# Autodesk Inventor assembly: schunk_with_gripper_fingers
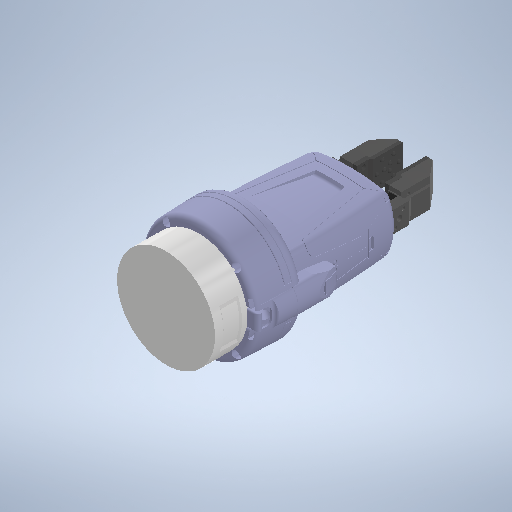
[picture p0: Inventor's stored thumbnail of the model, 512x512]
Saved by Autodesk Inventor 2025 (Build 290162010, 162A)
## iProperties
Created: 2024-08-06
Part Number: schunk_with_gripper_fingers
Document SubType Name: Assembly
Designer: caubeeluck
Author: caubeeluck
## Documents named in this file (21)
- D:\Projects\Archived\Misc\github\autoclean\AutoClean\cad_files\gripper\final_models\gripper_assembly_open\schunk_with_gripper_fingers.iam
- D:\Projects\Archived\Misc\github\autoclean\AutoClean\cad_files\gripper\final_models\gripper_assembly_open\schunk_with_gripper_fingers1.ipt
- D:\Projects\Archived\Misc\github\autoclean\AutoClean\cad_files\gripper\final_models\gripper_assembly_open\schunk_with_gripper_fingers2.ipt
- D:\Projects\Archived\Misc\github\autoclean\AutoClean\cad_files\gripper\final_models\gripper_assembly_open\schunk_with_gripper_fingers3.ipt
- D:\Projects\Archived\Misc\github\autoclean\AutoClean\cad_files\gripper\final_models\gripper_assembly_open\schunk_with_gripper_fingers4.ipt
- D:\Projects\Archived\Misc\github\autoclean\AutoClean\cad_files\gripper\final_models\gripper_assembly_open\schunk_with_gripper_fingers6.ipt
- D:\Projects\Archived\Misc\github\autoclean\AutoClean\cad_files\gripper\final_models\gripper_assembly_open\schunk_with_gripper_fingers7.ipt
- D:\Projects\Archived\Misc\github\autoclean\AutoClean\cad_files\gripper\final_models\gripper_assembly_open\schunk_with_gripper_fingers8.ipt
- D:\Projects\Archived\Misc\github\autoclean\AutoClean\cad_files\gripper\final_models\gripper_assembly_open\schunk_with_gripper_fingers9.ipt
- D:\Projects\Archived\Misc\github\autoclean\AutoClean\cad_files\gripper\final_models\gripper_assembly_open\schunk_with_gripper_fingers10.ipt
- D:\Projects\Archived\Misc\github\autoclean\AutoClean\cad_files\gripper\final_models\gripper_assembly_open\schunk_with_gripper_fingers11.ipt
- D:\Projects\Archived\Misc\github\autoclean\AutoClean\cad_files\gripper\final_models\gripper_assembly_open\schunk_with_gripper_fingers12.ipt
- D:\Projects\Archived\Misc\github\autoclean\AutoClean\cad_files\gripper\final_models\gripper_assembly_open\schunk_with_gripper_fingers13.ipt
- D:\Projects\Archived\Misc\github\autoclean\AutoClean\cad_files\gripper\final_models\gripper_assembly_open\schunk_with_gripper_fingers14.ipt
- D:\Projects\Archived\Misc\github\autoclean\AutoClean\cad_files\gripper\final_models\gripper_assembly_open\schunk_with_gripper_fingers15.ipt
- D:\Projects\Archived\Misc\github\autoclean\AutoClean\cad_files\gripper\final_models\gripper_assembly_open\schunk_with_gripper_fingers16.ipt
- D:\Projects\Archived\Misc\github\autoclean\AutoClean\cad_files\gripper\final_models\gripper_assembly_open\schunk_with_gripper_fingers17.ipt
- D:\Projects\Archived\Misc\github\autoclean\AutoClean\cad_files\gripper\final_models\gripper_assembly_open\schunk_with_gripper_fingers18.ipt
- D:\Projects\Archived\Misc\github\autoclean\AutoClean\cad_files\gripper\final_models\gripper_assembly_open\schunk_with_gripper_fingers19.ipt
- D:\Projects\Archived\Misc\github\autoclean\AutoClean\cad_files\gripper\final_models\gripper_assembly_open\schunk_with_gripper_fingers20.ipt
- D:\Projects\Archived\Misc\github\autoclean\AutoClean\cad_files\gripper\final_models\gripper_assembly_open\ur5_CAD24.ipt
## Components (20 placed, 20 different names)
1. schunk_with_gripper_fingers1:1 — Mate:1, Mate:2, Mate:3
2. schunk_with_gripper_fingers2:1
3. schunk_with_gripper_fingers3:1
4. schunk_with_gripper_fingers4:1
5. schunk_with_gripper_fingers6:1
6. schunk_with_gripper_fingers7:1
7. schunk_with_gripper_fingers8:1
8. schunk_with_gripper_fingers9:1
9. schunk_with_gripper_fingers10:1
10. schunk_with_gripper_fingers11:1
11. schunk_with_gripper_fingers12:1
12. schunk_with_gripper_fingers13:1
13. schunk_with_gripper_fingers14:1
14. schunk_with_gripper_fingers15:1
15. schunk_with_gripper_fingers16:1
16. schunk_with_gripper_fingers17:1
17. schunk_with_gripper_fingers18:1
18. schunk_with_gripper_fingers19:1
19. schunk_with_gripper_fingers20:1
20. ur5_CAD24:1 — Mate:1, Mate:2, Mate:3
## Relationships (3: Mate 3)
- Mate:1: schunk_with_gripper_fingers1:1 ↔ ur5_CAD24:1
- Mate:2: schunk_with_gripper_fingers1:1 ↔ ur5_CAD24:1
- Mate:3: schunk_with_gripper_fingers1:1 ↔ ur5_CAD24:1
